# Autodesk Inventor assembly: GE-12027
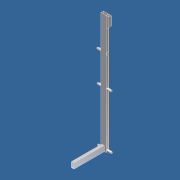
[picture p0: Inventor's stored thumbnail of the model, 180x180]
Saved by Autodesk Inventor 2012 (Build 160160000, 160)
## iProperties
Created: 2011-07-18
Part Number: GE-12027
Document SubType Name: Assembly
Designer: dfoster
Description: Hoop Upright, Right
Title: Hoop Upright, Right
Author: dfoster
## Documents named in this file (7)
- C:\Data Folder\FRC 2012 Field\Components\GE-12027.iam
- C:\Data Folder\FRC 2012 Field\Components\GE-12027-04.ipt
- C:\Data Folder\FRC 2012 Field\Components\GE-12027-03.ipt
- C:\Data Folder\FRC 2012 Field\Components\GE-12027-02.ipt
- C:\Data Folder\FRC 2012 Field\Components\GE-12027-01.ipt
- C:\Data Folder\FRC 2012 Field\Components\GE-12027-05.ipt
- C:\Data Folder\FRC 2012 Field\Components\GE-12027-06.ipt
## Components (10 placed, 6 different names)
1. GE-12027-01:1 — Flush:1, Flush:2, Mate:1, Mate:2, Flush:3, Mate:3, Flush:4, Mate:4, Flush:5, Flush:6, Flush:8, Mate:5, Flush:9, Mate:6, Flush:10, Mate:7, Mate:8, Flush:11, Mate:10, Mate:11, Mate:12, Flush:13, Flush:14, Flush:15
2. GE-12027-02:1 — Mate:2, Flush:3
3. GE-12027-02:2 — Mate:3, Flush:4
4. GE-12027-03:1 — Mate:4, Flush:5, Flush:6
5. GE-12027-04:1 — Flush:8, Mate:5
6. GE-12027-05:1 — Flush:9, Mate:6, Flush:10
7. GE-12027-06:1 — Mate:8, Mate:9, Flush:11, Flush:12, Mate:10
8. GE-12027-06:2 — Mate:7, Mate:9, Flush:12
9. GE-12027-06:3 — Mate:11, Mate:13, Flush:13, Flush:15
10. GE-12027-06:4 — Mate:12, Mate:13, Flush:14
## Relationships (27: Flush 14, Mate 13)
- Flush:1: GE-12027-01:1
- Flush:2: GE-12027-01:1
- Mate:1: GE-12027-01:1
- Mate:2: GE-12027-01:1 ↔ GE-12027-02:1
- Flush:3 (73.025 mm): GE-12027-01:1 ↔ GE-12027-02:1
- Mate:3: GE-12027-01:1 ↔ GE-12027-02:2
- Flush:4 (-66.675 mm): GE-12027-01:1 ↔ GE-12027-02:2
- Mate:4: GE-12027-01:1 ↔ GE-12027-03:1
- Flush:5: GE-12027-01:1 ↔ GE-12027-03:1
- Flush:6: GE-12027-01:1 ↔ GE-12027-03:1
- Flush:8 (-79.375 mm): GE-12027-01:1 ↔ GE-12027-04:1
- Mate:5: GE-12027-01:1 ↔ GE-12027-04:1
- Flush:9 (28.575 mm): GE-12027-01:1 ↔ GE-12027-05:1
- Mate:6: GE-12027-01:1 ↔ GE-12027-05:1
- Flush:10: GE-12027-01:1 ↔ GE-12027-05:1
- Mate:7: GE-12027-01:1 ↔ GE-12027-06:2
- Mate:8: GE-12027-01:1 ↔ GE-12027-06:1
- Mate:9 (34.925 mm): GE-12027-06:1 ↔ GE-12027-06:2
- Flush:11 (1.5875 mm): GE-12027-01:1 ↔ GE-12027-06:1
- Flush:12: GE-12027-06:1 ↔ GE-12027-06:2
- Mate:10 (-1228.725 mm): GE-12027-01:1 ↔ GE-12027-06:1
- Mate:11: GE-12027-01:1 ↔ GE-12027-06:3
- Mate:12: GE-12027-01:1 ↔ GE-12027-06:4
- Mate:13 (34.925 mm): GE-12027-06:3 ↔ GE-12027-06:4
- Flush:13: GE-12027-01:1 ↔ GE-12027-06:3
- Flush:14: GE-12027-01:1 ↔ GE-12027-06:4
- Flush:15 (1.5875 mm): GE-12027-01:1 ↔ GE-12027-06:3
